# Autodesk Inventor assembly: bts_asembly
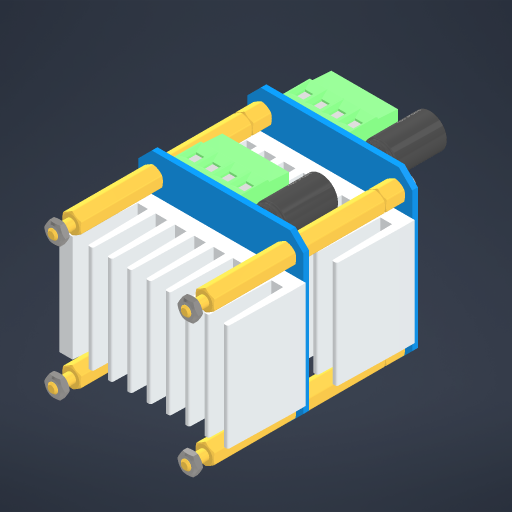
[picture p0: Inventor's stored thumbnail of the model, 512x512]
Saved by Autodesk Inventor 2024 (Build 280153000, 153)
## iProperties
Created: 2023-05-16
Part Number: bts_asembly
Document SubType Name: Assembly
Designer: user
Author: user
## Documents named in this file (6)
- D:\Docs\Robot\3d\electronics\bts_asembly.iam
- D:\Docs\Robot\3d\electronics\BTS7960\BTS7960.iam
- D:\Docs\Robot\3d\default_components\PCHSN\PCHSN-25.ipt
- D:\Docs\Robot\3d\default_components\PCHSN\PCHSN-6.ipt
- C:\Users\user\Documents\Inventor\Content Center Files\R2024\ru-RU\DIN 7985 (H)\DIN 7985 (H) - M3x6-H.ipt
- C:\Users\user\Documents\Inventor\Content Center Files\R2024\ru-RU\DIN 934\DIN 934 - M3 x 0,5.ipt
## Components (22 placed, 5 different names)
1. BTS7960:1 [sub-assembly] — Вставка:3, Вставка:4, Вставка:11, Вставка:12, Вставка:13, Вставка:14, Совмещение:1, Заподлицо:1, Совмещение:2
2. BTS7960:2 [sub-assembly] — Вставка:5, Вставка:6, Вставка:9, Вставка:10, Вставка:15, Вставка:16, Вставка:17, Вставка:18
3. PCHSN-25:2 — Вставка:2, Вставка:4
4. PCHSN-25:3 — Вставка:1, Вставка:3
5. PCHSN-6:1 — Вставка:1, Вставка:6
6. PCHSN-6:2 — Вставка:2, Вставка:5
7. PCHSN-6:3 — Вставка:8, Вставка:9
8. PCHSN-25:4 — Вставка:7
9. PCHSN-25:5 — Вставка:8
10. PCHSN-6:4 — Вставка:7, Вставка:10
11. PCHSN-25:6 — Вставка:11, Вставка:19
12. PCHSN-25:7 — Вставка:13, Вставка:22
13. PCHSN-25:8 — Вставка:14, Вставка:20
14. PCHSN-25:9 — Вставка:12, Вставка:21
15. DIN 7985 (H) M3x6-H:1 — Вставка:17
16. DIN 7985 (H) M3x6-H:2 — Вставка:18
17. DIN 7985 (H) M3x6-H:3 — Вставка:16
18. DIN 7985 (H) M3x6-H:4 — Вставка:15
19. DIN 934 - заменено на DIN EN 24032/28673/28674 M3:1 — Вставка:22
20. DIN 934 - заменено на DIN EN 24032/28673/28674 M3:2 — Вставка:21
21. DIN 934 - заменено на DIN EN 24032/28673/28674 M3:3 — Вставка:20
22. DIN 934 - заменено на DIN EN 24032/28673/28674 M3:4 — Вставка:19
## Relationships (25: Insert 22, Mate 2, Flush 1)
- Вставка:1 [Insert]: PCHSN-25:3 ↔ PCHSN-6:1
- Вставка:2 [Insert]: PCHSN-25:2 ↔ PCHSN-6:2
- Вставка:3 [Insert]: BTS7960:1 ↔ PCHSN-25:3
- Вставка:4 [Insert]: BTS7960:1 ↔ PCHSN-25:2
- Вставка:5 [Insert]: BTS7960:2 ↔ PCHSN-6:2
- Вставка:6 [Insert]: BTS7960:2 ↔ PCHSN-6:1
- Вставка:7 [Insert]: PCHSN-25:4 ↔ PCHSN-6:4
- Вставка:8 [Insert]: PCHSN-6:3 ↔ PCHSN-25:5
- Вставка:9 [Insert]: BTS7960:2 ↔ PCHSN-6:3
- Вставка:10 [Insert]: BTS7960:2 ↔ PCHSN-6:4
- Вставка:11 [Insert]: BTS7960:1 ↔ PCHSN-25:6
- Вставка:12 [Insert]: BTS7960:1 ↔ PCHSN-25:9
- Вставка:13 [Insert]: BTS7960:1 ↔ PCHSN-25:7
- Вставка:14 [Insert]: BTS7960:1 ↔ PCHSN-25:8
- Вставка:15 [Insert]: BTS7960:2 ↔ DIN 7985 (H) M3x6-H:4
- Вставка:16 [Insert]: BTS7960:2 ↔ DIN 7985 (H) M3x6-H:3
- Вставка:17 [Insert]: BTS7960:2 ↔ DIN 7985 (H) M3x6-H:1
- Вставка:18 [Insert]: BTS7960:2 ↔ DIN 7985 (H) M3x6-H:2
- Вставка:19 [Insert] (3 mm): PCHSN-25:6 ↔ DIN 934 - заменено на DIN EN 24032/28673/28674 M3:4
- Вставка:20 [Insert] (3 mm): PCHSN-25:8 ↔ DIN 934 - заменено на DIN EN 24032/28673/28674 M3:3
- Вставка:21 [Insert] (3 mm): PCHSN-25:9 ↔ DIN 934 - заменено на DIN EN 24032/28673/28674 M3:2
- Вставка:22 [Insert] (3 mm): PCHSN-25:7 ↔ DIN 934 - заменено на DIN EN 24032/28673/28674 M3:1
- Совмещение:1 [Mate]: BTS7960:1
- Заподлицо:1 [Flush]: BTS7960:1
- Совмещение:2 [Mate]: BTS7960:1
